# Autodesk Inventor assembly: 出力ピンユニット
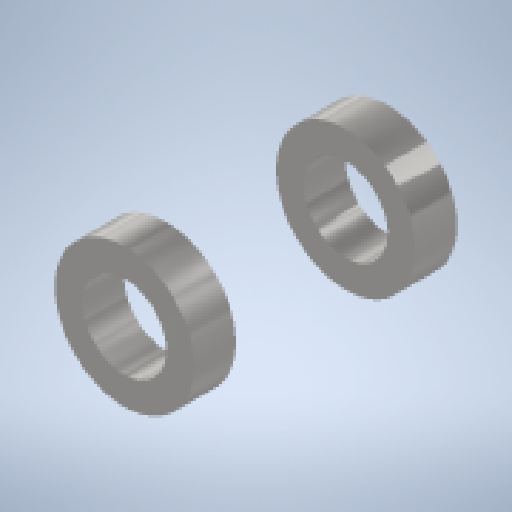
[picture p0: Inventor's stored thumbnail of the model, 512x512]
Saved by Autodesk Inventor 2024 (Build 280153000, 153)
## iProperties
Created: 2023-05-29
Part Number: 出力ピンユニット
Document SubType Name: Assembly
Designer: yuta2
Author: yuta2
## Documents named in this file (3)
- C:\Users\yuta2\Documents\Inventor\mokemoke2023\サイクロイド減速機_大型\出力ピンユニット.iam
- C:\Users\yuta2\Documents\Inventor\mokemoke2023\ベアリング\676ZZ.ipt
- C:\Users\yuta2\Documents\Inventor\mokemoke2023\サイクロイド減速機_大型\出力ピン.ipt
## Components (3 placed, 2 different names)
1. 676ZZ:1 — 回転:1, 回転:2
2. 676ZZ:2 — 回転:2
3. 出力ピン:1 — 回転:1
## Relationships (2: RevoluteJoint 2)
- 回転:1 [RevoluteJoint] (-6.5 mm): 676ZZ:1 ↔ 出力ピン:1
- 回転:2 [RevoluteJoint] (-2 mm): 676ZZ:1 ↔ 676ZZ:2
